# Autodesk Inventor assembly: #Spindexer
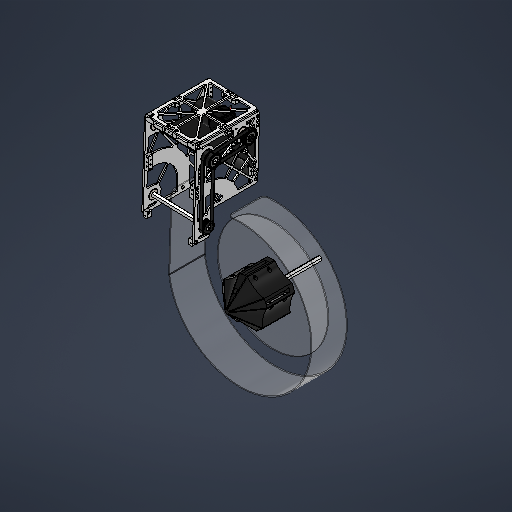
[picture p0: Inventor's stored thumbnail of the model, 512x512]
Saved by Autodesk Inventor 2026.1 (Build 301233020, 233B)
## iProperties
Created: 2026-02-05
Part Number: #Spindexer
Document SubType Name: Assembly
Designer: Owen L
Mass: 3778.08 g
Surface Area: 11708.6 cm^2
Volume: 3965.25 cm^3
Density: 0.952797 g/cm^3
Author: Owen L
## Documents named in this file (30)
- C:\Users\Owen\Documents\GitHub\2026-Robot-Mechanical\Spindexer\#Spindexer.iam
- C:\Users\Owen\Documents\GitHub\2026-Robot-Mechanical\Spindexer\3DPRINT,HUB.ipt
- C:\Users\Owen\Documents\GitHub\2026-Robot-Mechanical\Spindexer\3DPRINT,HUB,CONE.ipt
- C:\Users\Owen\Documents\GitHub\2026-Robot-Mechanical\Spindexer\PLATE,WALL.ipt
- C:\Users\Owen\Documents\GitHub\2026-Robot-Mechanical\Spindexer\PLATE,BOTTOM.ipt
- C:\Users\Owen\Documents\GitHub\2026-Robot-Mechanical\Spindexer\STOCK,HEX,SHAFT,HUB.ipt
- C:\Users\Owen\Documents\GitHub\2026-Robot-Mechanical\Spindexer\TEMP,BASE-SKETCH,TANGENT-OUT.ipt
- C:\Users\Owen\Documents\GitHub\2026-Robot-Mechanical\Spindexer\PLATE,KICKER,OUTSIDE.ipt
- C:\Users\Owen\Documents\GitHub\2026-Robot-Mechanical\Spindexer\3DPRINT,KICKER,RAMP.ipt
- C:\Users\Owen\Documents\GitHub\2026-Robot-Mechanical\Spindexer\PLATE,KICKER,INSIDE.ipt
- C:\Users\Owen\Documents\GitHub\2026-Robot-Mechanical\Spindexer\STOCK,HEX,SHAFT,KICKER,FRONT.ipt
- C:\Users\Owen\Documents\GitHub\2026-Robot-Mechanical\Spindexer\STOCK,HEX,SHAFT,KICKER,BACK.ipt
- C:\Users\Owen\Documents\GitHub\2026-Robot-Mechanical\#1_CAD Library\Power Transmission\Bearings\PURCHASED,HEX_BEARING.ipt
- C:\Users\Owen\Documents\GitHub\2026-Robot-Mechanical\#1_CAD Library\Power Transmission\VersaPlanetary\GEARBOX,VERSAPLANETARY,SINGLE-STAGE,HEX-SHAFT,0.5IN.ipt
- C:\Users\Owen\Documents\GitHub\2026-Robot-Mechanical\#1_CAD Library\Power Transmission\VersaPlanetary\ADAPTER,CIM-NEO,VERSAPLANETARY.ipt
- C:\Users\Owen\Documents\GitHub\2026-Robot-Mechanical\#1_CAD Library\Motors\MOTOR,REV,NEO,V1-1.ipt
- C:\Users\Owen\Documents\GitHub\2026-Robot-Mechanical\Spindexer\PLATE,NUT-BLOCK,3-LONG.ipt
- C:\Users\Owen\Documents\GitHub\2026-Robot-Mechanical\Spindexer\PLATE,NUT-BLOCK,2-LONG.ipt
- C:\Users\Owen\Documents\GitHub\2026-Robot-Mechanical\Spindexer\PLATE,NUT-BLOCK,1-LONG.ipt
- C:\Users\Owen\Documents\GitHub\2026-Robot-Mechanical\#1_CAD Library\Electronics\CONTROLS,SPARK_MAX.ipt
- C:\Users\Owen\Documents\GitHub\2026-Robot-Mechanical\Spindexer\3DPRINT,SPARK_MAX,MOUNT.ipt
- C:\Users\Owen\Documents\GitHub\2026-Robot-Mechanical\Spindexer\PLATE,KICKER,BACK.ipt
- C:\Users\Owen\Documents\GitHub\2026-Robot-Mechanical\Spindexer\PLATE,NUT-BLOCK,L-SHAPE.ipt
- C:\Users\Owen\Documents\GitHub\2026-Robot-Mechanical\Spindexer\3DPRINTED,PULLEY,21T,9mm.ipt
- C:\Users\Owen\Documents\GitHub\2026-Robot-Mechanical\#1_CAD Library\Power Transmission\Pulleys\PURCHASED,HTD5mm,24T,PULLEY.ipt
- C:\Users\Owen\Documents\GitHub\2026-Robot-Mechanical\Spindexer\STANDIN,BELT,70T,HTD5mm.ipt
- C:\Users\Owen\Documents\GitHub\2026-Robot-Mechanical\Spindexer\STANDIN,BELT,100T,HTD5mm.ipt
- C:\Users\Owen\Documents\GitHub\2026-Robot-Mechanical\#1_CAD Library\Building Materials\Fasteners\Bolts\PURCHASED,10-32x0.5in,BUTTONHEAD,BOLT.ipt
- C:\Users\Owen\Documents\GitHub\2026-Robot-Mechanical\#1_CAD Library\Building Materials\Fasteners\Nuts\PURCHASED,NYLOCK,10-32,NUT.ipt
- C:\Users\Owen\Documents\GitHub\2026-Robot-Mechanical\#1_CAD Library\Building Materials\Fasteners\Bolts\PURCHASED,10-32x0.625in,BUTTONHEAD,BOLT.ipt
## Components (90 placed, 29 different names)
1. 3DPRINT,HUB:1 — Mate:11, Mate:12, Mate:13, Mate:15, Mate:16, Mate:17, Flush:2, Mate:18, Mate:19, Mate:20
2. 3DPRINT,HUB,CONE:1 — Mate:11, Mate:12, Mate:13
3. PLATE,WALL:1 — Mate:32, Flush:7, Flush:8, Mate:42, Mate:43
4. PLATE,BOTTOM:1 — Mate:18, Mate:19, Mate:20, Mate:32, Flush:7
5. STOCK,HEX,SHAFT,HUB:1 — Mate:16, Mate:17, Flush:2
6. TEMP,BASE-SKETCH,TANGENT-OUT:1
7. PLATE,KICKER,OUTSIDE:1 — Mate:22, Mate:23, Mate:24, Mate:25, Flush:3, Flush:4, Flush:8, Insert:1, Insert:4, Mate:34, Mate:35, Mate:42, Insert:7, Insert:8, Insert:9, Insert:10, Insert:13, Insert:19, Insert:20, Flush:12, Mate:43, Insert:23, Insert:24, Insert:34, Insert:35, Insert:36, Insert:37, Insert:38, Insert:39, Insert:40, Insert:41, Insert:42, Insert:43, Insert:44, Insert:45, Insert:46, Insert:47, Insert:48, Insert:49, Insert:50, Insert:79, Insert:80, Insert:81, Insert:82
8. 3DPRINT,KICKER,RAMP:1 — Mate:22, Mate:23, Mate:24
9. PLATE,KICKER,INSIDE:1 — Mate:25, Flush:3, Flush:4, Insert:2, Insert:3, Mate:39, Mate:40, Mate:41, Insert:6, Insert:14, Insert:17, Insert:18, Insert:21, Insert:22, Insert:31, Insert:32, Insert:33, Mate:48, Mate:52, Insert:61, Insert:62, Insert:63, Insert:64, Insert:65, Insert:66, Insert:67, Insert:68, Insert:69, Insert:70, Insert:71, Insert:72, Insert:73, Insert:74, Insert:75, Insert:76, Insert:77, Insert:78
10. STOCK,HEX,SHAFT,KICKER,FRONT:1 — Mate:34, Mate:45, Flush:15
11. STOCK,HEX,SHAFT,KICKER,BACK:1 — Mate:35, Mate:46, Mate:47, Flush:14
12. PURCHASED,HEX_BEARING:1 — Insert:1, Flush:15
13. PURCHASED,HEX_BEARING:2 — Insert:2, Mate:50
14. PURCHASED,HEX_BEARING:3 — Insert:3, Mate:49
15. PURCHASED,HEX_BEARING:4 — Insert:4, Flush:14
16. GEARBOX,VERSAPLANETARY,SINGLE-STAGE,HEX-SHAFT,0.5IN:1 — Mate:36, Mate:37, Mate:38, Mate:39, Mate:40, Mate:41, Mate:53
17. ADAPTER,CIM-NEO,VERSAPLANETARY:1 — Mate:36, Mate:37, Mate:38, Insert:5
18. MOTOR,REV,NEO,V1-1:1 — Insert:5
19. PLATE,NUT-BLOCK,3-LONG:1 — Insert:6
20. PLATE,NUT-BLOCK,3-LONG:2 — Insert:9, Insert:10
21. PLATE,NUT-BLOCK,3-LONG:3 — Insert:7, Insert:8
22. PLATE,NUT-BLOCK,1-LONG:1 — Insert:13, Flush:11, Flush:12
23. PLATE,NUT-BLOCK,1-LONG:2 — Insert:14, Flush:11
24. PLATE,NUT-BLOCK,3-LONG:4 — Insert:17, Insert:18
25. PLATE,NUT-BLOCK,3-LONG:5 — Insert:19, Insert:20
26. CONTROLS,SPARK_MAX:1
27. 3DPRINT,SPARK_MAX,MOUNT:1
28. PLATE,KICKER,BACK:1 — Mate:44, Insert:25, Insert:26, Insert:27, Insert:28, Insert:29, Insert:30, Insert:51, Insert:52, Insert:53, Insert:54, Insert:55, Insert:56, Insert:57, Insert:58, Insert:59, Insert:60
29. PLATE,NUT-BLOCK,2-LONG:2 — Insert:21, Insert:22, Mate:44, Insert:26
30. PLATE,NUT-BLOCK,2-LONG:3 — Insert:23, Insert:24, Insert:25
31. PLATE,NUT-BLOCK,3-LONG:6 — Insert:27, Insert:28
32. PLATE,NUT-BLOCK,3-LONG:7 — Insert:29, Insert:30
33. PLATE,NUT-BLOCK,3-LONG:8 — Insert:31, Insert:32
34. PLATE,NUT-BLOCK,L-SHAPE:1 — Insert:33
35. PLATE,NUT-BLOCK,L-SHAPE:2 — Insert:34
36. 3DPRINTED,PULLEY,21T,9mm:1 — Mate:46, Mate:49, Mate:51, Mate:55, Mate:58
37. 3DPRINTED,PULLEY,21T,9mm:2 — Mate:45, Mate:50, Mate:54
38. PURCHASED,HEX_BEARING:5 — Mate:52, Mate:53
39. PURCHASED,HTD5mm,24T,PULLEY:1 — Mate:47, Mate:51, Flush:13, Mate:57
40. PURCHASED,HTD5mm,24T,PULLEY:2 — Mate:48, Flush:13, Mate:56
41. STANDIN,BELT,70T,HTD5mm:1 — Mate:56, Mate:57
42. STANDIN,BELT,100T,HTD5mm:1 — Mate:54, Mate:55, Mate:58
43. PURCHASED,10-32x0.5in,BUTTONHEAD,BOLT:1 — Insert:48
44. PURCHASED,NYLOCK,10-32,NUT:1 — Insert:81
45. PURCHASED,10-32x0.625in,BUTTONHEAD,BOLT:1 — Insert:35
46. PURCHASED,10-32x0.625in,BUTTONHEAD,BOLT:2 — Insert:36
47. PURCHASED,10-32x0.625in,BUTTONHEAD,BOLT:3 — Insert:37
48. PURCHASED,10-32x0.625in,BUTTONHEAD,BOLT:4 — Insert:38
49. PURCHASED,10-32x0.625in,BUTTONHEAD,BOLT:5 — Insert:39
50. PURCHASED,10-32x0.625in,BUTTONHEAD,BOLT:6 — Insert:40
51. PURCHASED,10-32x0.625in,BUTTONHEAD,BOLT:7 — Insert:41
52. PURCHASED,10-32x0.625in,BUTTONHEAD,BOLT:8 — Insert:42
53. PURCHASED,10-32x0.625in,BUTTONHEAD,BOLT:9 — Insert:43
54. PURCHASED,10-32x0.625in,BUTTONHEAD,BOLT:10 — Insert:44
55. PURCHASED,10-32x0.625in,BUTTONHEAD,BOLT:11 — Insert:45
56. PURCHASED,10-32x0.625in,BUTTONHEAD,BOLT:12 — Insert:46
57. PURCHASED,10-32x0.625in,BUTTONHEAD,BOLT:13 — Insert:47
58. PURCHASED,10-32x0.625in,BUTTONHEAD,BOLT:14 — Insert:51
59. PURCHASED,10-32x0.625in,BUTTONHEAD,BOLT:15 — Insert:52
60. PURCHASED,10-32x0.625in,BUTTONHEAD,BOLT:16 — Insert:53
61. PURCHASED,10-32x0.625in,BUTTONHEAD,BOLT:17 — Insert:54
62. PURCHASED,10-32x0.625in,BUTTONHEAD,BOLT:18 — Insert:55
63. PURCHASED,10-32x0.5in,BUTTONHEAD,BOLT:2 — Insert:49
64. PURCHASED,10-32x0.5in,BUTTONHEAD,BOLT:3 — Insert:50
65. PURCHASED,10-32x0.625in,BUTTONHEAD,BOLT:19 — Insert:59
66. PURCHASED,10-32x0.625in,BUTTONHEAD,BOLT:20 — Insert:58
67. PURCHASED,10-32x0.625in,BUTTONHEAD,BOLT:21 — Insert:56
68. PURCHASED,10-32x0.625in,BUTTONHEAD,BOLT:22 — Insert:60
69. PURCHASED,10-32x0.625in,BUTTONHEAD,BOLT:23 — Insert:57
70. PURCHASED,10-32x0.625in,BUTTONHEAD,BOLT:24 — Insert:61
71. PURCHASED,10-32x0.625in,BUTTONHEAD,BOLT:25 — Insert:62
72. PURCHASED,10-32x0.625in,BUTTONHEAD,BOLT:26 — Insert:63
73. PURCHASED,10-32x0.625in,BUTTONHEAD,BOLT:27 — Insert:64
74. PURCHASED,10-32x0.625in,BUTTONHEAD,BOLT:28 — Insert:65
75. PURCHASED,10-32x0.625in,BUTTONHEAD,BOLT:29 — Insert:66
76. PURCHASED,10-32x0.625in,BUTTONHEAD,BOLT:30 — Insert:67
77. PURCHASED,10-32x0.625in,BUTTONHEAD,BOLT:31 — Insert:68
78. PURCHASED,10-32x0.625in,BUTTONHEAD,BOLT:32 — Insert:69
79. PURCHASED,10-32x0.625in,BUTTONHEAD,BOLT:33 — Insert:70
80. PURCHASED,10-32x0.625in,BUTTONHEAD,BOLT:34 — Insert:73
81. PURCHASED,10-32x0.625in,BUTTONHEAD,BOLT:35 — Insert:72
82. PURCHASED,10-32x0.625in,BUTTONHEAD,BOLT:36 — Insert:71
83. PURCHASED,10-32x0.5in,BUTTONHEAD,BOLT:4 — Insert:74
84. PURCHASED,10-32x0.5in,BUTTONHEAD,BOLT:5 — Insert:76
85. PURCHASED,10-32x0.5in,BUTTONHEAD,BOLT:6 — Insert:75
86. PURCHASED,10-32x0.5in,BUTTONHEAD,BOLT:7 — Insert:77
87. PURCHASED,10-32x0.5in,BUTTONHEAD,BOLT:8 — Insert:78
88. PURCHASED,10-32x0.5in,BUTTONHEAD,BOLT:9 — Insert:79
89. PURCHASED,10-32x0.5in,BUTTONHEAD,BOLT:10 — Insert:80
90. PURCHASED,NYLOCK,10-32,NUT:2 — Insert:82
## Relationships (127: Insert 78, Mate 39, Flush 10)
- Mate:11: 3DPRINT,HUB:1 ↔ 3DPRINT,HUB,CONE:1
- Mate:12: 3DPRINT,HUB:1 ↔ 3DPRINT,HUB,CONE:1
- Mate:13: 3DPRINT,HUB:1 ↔ 3DPRINT,HUB,CONE:1
- Mate:15: 3DPRINT,HUB:1
- Mate:16: 3DPRINT,HUB:1 ↔ STOCK,HEX,SHAFT,HUB:1
- Mate:17: 3DPRINT,HUB:1 ↔ STOCK,HEX,SHAFT,HUB:1
- Flush:2 (-12.7 mm): 3DPRINT,HUB:1 ↔ STOCK,HEX,SHAFT,HUB:1
- Mate:18: 3DPRINT,HUB:1 ↔ PLATE,BOTTOM:1
- Mate:19: 3DPRINT,HUB:1 ↔ PLATE,BOTTOM:1
- Mate:20: 3DPRINT,HUB:1 ↔ PLATE,BOTTOM:1
- Mate:22: PLATE,KICKER,OUTSIDE:1 ↔ 3DPRINT,KICKER,RAMP:1
- Mate:23: PLATE,KICKER,OUTSIDE:1 ↔ 3DPRINT,KICKER,RAMP:1
- Mate:24: PLATE,KICKER,OUTSIDE:1 ↔ 3DPRINT,KICKER,RAMP:1
- Mate:25 (158.75 mm): PLATE,KICKER,OUTSIDE:1 ↔ PLATE,KICKER,INSIDE:1
- Flush:3: PLATE,KICKER,OUTSIDE:1 ↔ PLATE,KICKER,INSIDE:1
- Flush:4: PLATE,KICKER,OUTSIDE:1 ↔ PLATE,KICKER,INSIDE:1
- Mate:32: PLATE,WALL:1 ↔ PLATE,BOTTOM:1
- Flush:7 (-6.35 mm): PLATE,WALL:1 ↔ PLATE,BOTTOM:1
- Flush:8: PLATE,WALL:1 ↔ PLATE,KICKER,OUTSIDE:1
- Insert:1: PLATE,KICKER,OUTSIDE:1 ↔ PURCHASED,HEX_BEARING:1
- Insert:2: PLATE,KICKER,INSIDE:1 ↔ PURCHASED,HEX_BEARING:2
- Insert:3: PLATE,KICKER,INSIDE:1 ↔ PURCHASED,HEX_BEARING:3
- Insert:4: PLATE,KICKER,OUTSIDE:1 ↔ PURCHASED,HEX_BEARING:4
- Mate:34: PLATE,KICKER,OUTSIDE:1 ↔ STOCK,HEX,SHAFT,KICKER,FRONT:1
- Mate:35: PLATE,KICKER,OUTSIDE:1 ↔ STOCK,HEX,SHAFT,KICKER,BACK:1
- Mate:36: GEARBOX,VERSAPLANETARY,SINGLE-STAGE,HEX-SHAFT,0.5IN:1 ↔ ADAPTER,CIM-NEO,VERSAPLANETARY:1
- Mate:37: GEARBOX,VERSAPLANETARY,SINGLE-STAGE,HEX-SHAFT,0.5IN:1 ↔ ADAPTER,CIM-NEO,VERSAPLANETARY:1
- Mate:38: GEARBOX,VERSAPLANETARY,SINGLE-STAGE,HEX-SHAFT,0.5IN:1 ↔ ADAPTER,CIM-NEO,VERSAPLANETARY:1
- Insert:5: ADAPTER,CIM-NEO,VERSAPLANETARY:1 ↔ MOTOR,REV,NEO,V1-1:1
- Mate:39: PLATE,KICKER,INSIDE:1 ↔ GEARBOX,VERSAPLANETARY,SINGLE-STAGE,HEX-SHAFT,0.5IN:1
- Mate:40: PLATE,KICKER,INSIDE:1 ↔ GEARBOX,VERSAPLANETARY,SINGLE-STAGE,HEX-SHAFT,0.5IN:1
- Mate:41: PLATE,KICKER,INSIDE:1 ↔ GEARBOX,VERSAPLANETARY,SINGLE-STAGE,HEX-SHAFT,0.5IN:1
- Mate:42: PLATE,WALL:1 ↔ PLATE,KICKER,OUTSIDE:1
- Insert:6: PLATE,KICKER,INSIDE:1 ↔ PLATE,NUT-BLOCK,3-LONG:1
- Insert:7: PLATE,KICKER,OUTSIDE:1 ↔ PLATE,NUT-BLOCK,3-LONG:3
- Insert:8: PLATE,KICKER,OUTSIDE:1 ↔ PLATE,NUT-BLOCK,3-LONG:3
- Insert:9: PLATE,KICKER,OUTSIDE:1 ↔ PLATE,NUT-BLOCK,3-LONG:2
- Insert:10: PLATE,KICKER,OUTSIDE:1 ↔ PLATE,NUT-BLOCK,3-LONG:2
- Insert:13: PLATE,KICKER,OUTSIDE:1 ↔ PLATE,NUT-BLOCK,1-LONG:1
- Insert:14: PLATE,KICKER,INSIDE:1 ↔ PLATE,NUT-BLOCK,1-LONG:2
- Insert:17: PLATE,KICKER,INSIDE:1 ↔ PLATE,NUT-BLOCK,3-LONG:4
- Insert:18: PLATE,KICKER,INSIDE:1 ↔ PLATE,NUT-BLOCK,3-LONG:4
- Insert:19: PLATE,KICKER,OUTSIDE:1 ↔ PLATE,NUT-BLOCK,3-LONG:5
- Insert:20: PLATE,KICKER,OUTSIDE:1 ↔ PLATE,NUT-BLOCK,3-LONG:5
- Flush:11: PLATE,NUT-BLOCK,1-LONG:1 ↔ PLATE,NUT-BLOCK,1-LONG:2
- Flush:12: PLATE,KICKER,OUTSIDE:1 ↔ PLATE,NUT-BLOCK,1-LONG:1
- Mate:43 (-25.4 mm): PLATE,WALL:1 ↔ PLATE,KICKER,OUTSIDE:1
- Insert:21: PLATE,KICKER,INSIDE:1 ↔ PLATE,NUT-BLOCK,2-LONG:2
- Insert:22: PLATE,KICKER,INSIDE:1 ↔ PLATE,NUT-BLOCK,2-LONG:2
- Insert:23: PLATE,KICKER,OUTSIDE:1 ↔ PLATE,NUT-BLOCK,2-LONG:3
- Insert:24: PLATE,KICKER,OUTSIDE:1 ↔ PLATE,NUT-BLOCK,2-LONG:3
- Mate:44: PLATE,KICKER,BACK:1 ↔ PLATE,NUT-BLOCK,2-LONG:2
- Insert:25: PLATE,KICKER,BACK:1 ↔ PLATE,NUT-BLOCK,2-LONG:3
- Insert:26: PLATE,KICKER,BACK:1 ↔ PLATE,NUT-BLOCK,2-LONG:2
- Insert:27: PLATE,KICKER,BACK:1 ↔ PLATE,NUT-BLOCK,3-LONG:6
- Insert:28: PLATE,KICKER,BACK:1 ↔ PLATE,NUT-BLOCK,3-LONG:6
- Insert:29: PLATE,KICKER,BACK:1 ↔ PLATE,NUT-BLOCK,3-LONG:7
- Insert:30: PLATE,KICKER,BACK:1 ↔ PLATE,NUT-BLOCK,3-LONG:7
- Insert:31: PLATE,KICKER,INSIDE:1 ↔ PLATE,NUT-BLOCK,3-LONG:8
- Insert:32: PLATE,KICKER,INSIDE:1 ↔ PLATE,NUT-BLOCK,3-LONG:8
- Insert:33: PLATE,KICKER,INSIDE:1 ↔ PLATE,NUT-BLOCK,L-SHAPE:1
- Insert:34: PLATE,KICKER,OUTSIDE:1 ↔ PLATE,NUT-BLOCK,L-SHAPE:2
- Mate:45: STOCK,HEX,SHAFT,KICKER,FRONT:1 ↔ 3DPRINTED,PULLEY,21T,9mm:2
- Mate:46: STOCK,HEX,SHAFT,KICKER,BACK:1 ↔ 3DPRINTED,PULLEY,21T,9mm:1
- Mate:47: STOCK,HEX,SHAFT,KICKER,BACK:1 ↔ PURCHASED,HTD5mm,24T,PULLEY:1
- Mate:48: PLATE,KICKER,INSIDE:1 ↔ PURCHASED,HTD5mm,24T,PULLEY:2
- Mate:49: PURCHASED,HEX_BEARING:3 ↔ 3DPRINTED,PULLEY,21T,9mm:1
- Mate:50: PURCHASED,HEX_BEARING:2 ↔ 3DPRINTED,PULLEY,21T,9mm:2
- Mate:51: 3DPRINTED,PULLEY,21T,9mm:1 ↔ PURCHASED,HTD5mm,24T,PULLEY:1
- Flush:13: PURCHASED,HTD5mm,24T,PULLEY:1 ↔ PURCHASED,HTD5mm,24T,PULLEY:2
- Flush:14: STOCK,HEX,SHAFT,KICKER,BACK:1 ↔ PURCHASED,HEX_BEARING:4
- Flush:15: STOCK,HEX,SHAFT,KICKER,FRONT:1 ↔ PURCHASED,HEX_BEARING:1
- Mate:52: PLATE,KICKER,INSIDE:1 ↔ PURCHASED,HEX_BEARING:5
- Mate:53: GEARBOX,VERSAPLANETARY,SINGLE-STAGE,HEX-SHAFT,0.5IN:1 ↔ PURCHASED,HEX_BEARING:5
- Mate:54: 3DPRINTED,PULLEY,21T,9mm:2 ↔ STANDIN,BELT,100T,HTD5mm:1
- Mate:55: 3DPRINTED,PULLEY,21T,9mm:1 ↔ STANDIN,BELT,100T,HTD5mm:1
- Mate:56: PURCHASED,HTD5mm,24T,PULLEY:2 ↔ STANDIN,BELT,70T,HTD5mm:1
- Mate:57: PURCHASED,HTD5mm,24T,PULLEY:1 ↔ STANDIN,BELT,70T,HTD5mm:1
- Mate:58: 3DPRINTED,PULLEY,21T,9mm:1 ↔ STANDIN,BELT,100T,HTD5mm:1
- Insert:35: PLATE,KICKER,OUTSIDE:1 ↔ PURCHASED,10-32x0.625in,BUTTONHEAD,BOLT:1
- Insert:36: PLATE,KICKER,OUTSIDE:1 ↔ PURCHASED,10-32x0.625in,BUTTONHEAD,BOLT:2
- Insert:37: PLATE,KICKER,OUTSIDE:1 ↔ PURCHASED,10-32x0.625in,BUTTONHEAD,BOLT:3
- Insert:38: PLATE,KICKER,OUTSIDE:1 ↔ PURCHASED,10-32x0.625in,BUTTONHEAD,BOLT:4
- Insert:39: PLATE,KICKER,OUTSIDE:1 ↔ PURCHASED,10-32x0.625in,BUTTONHEAD,BOLT:5
- Insert:40: PLATE,KICKER,OUTSIDE:1 ↔ PURCHASED,10-32x0.625in,BUTTONHEAD,BOLT:6
- Insert:41: PLATE,KICKER,OUTSIDE:1 ↔ PURCHASED,10-32x0.625in,BUTTONHEAD,BOLT:7
- Insert:42: PLATE,KICKER,OUTSIDE:1 ↔ PURCHASED,10-32x0.625in,BUTTONHEAD,BOLT:8
- Insert:43: PLATE,KICKER,OUTSIDE:1 ↔ PURCHASED,10-32x0.625in,BUTTONHEAD,BOLT:9
- Insert:44: PLATE,KICKER,OUTSIDE:1 ↔ PURCHASED,10-32x0.625in,BUTTONHEAD,BOLT:10
- Insert:45: PLATE,KICKER,OUTSIDE:1 ↔ PURCHASED,10-32x0.625in,BUTTONHEAD,BOLT:11
- Insert:46: PLATE,KICKER,OUTSIDE:1 ↔ PURCHASED,10-32x0.625in,BUTTONHEAD,BOLT:12
- Insert:47: PLATE,KICKER,OUTSIDE:1 ↔ PURCHASED,10-32x0.625in,BUTTONHEAD,BOLT:13
- Insert:48: PLATE,KICKER,OUTSIDE:1 ↔ PURCHASED,10-32x0.5in,BUTTONHEAD,BOLT:1
- Insert:49: PLATE,KICKER,OUTSIDE:1 ↔ PURCHASED,10-32x0.5in,BUTTONHEAD,BOLT:2
- Insert:50: PLATE,KICKER,OUTSIDE:1 ↔ PURCHASED,10-32x0.5in,BUTTONHEAD,BOLT:3
- Insert:51: PLATE,KICKER,BACK:1 ↔ PURCHASED,10-32x0.625in,BUTTONHEAD,BOLT:14
- Insert:52: PLATE,KICKER,BACK:1 ↔ PURCHASED,10-32x0.625in,BUTTONHEAD,BOLT:15
- Insert:53: PLATE,KICKER,BACK:1 ↔ PURCHASED,10-32x0.625in,BUTTONHEAD,BOLT:16
- Insert:54: PLATE,KICKER,BACK:1 ↔ PURCHASED,10-32x0.625in,BUTTONHEAD,BOLT:17
- Insert:55: PLATE,KICKER,BACK:1 ↔ PURCHASED,10-32x0.625in,BUTTONHEAD,BOLT:18
- Insert:56: PLATE,KICKER,BACK:1 ↔ PURCHASED,10-32x0.625in,BUTTONHEAD,BOLT:21
- Insert:57: PLATE,KICKER,BACK:1 ↔ PURCHASED,10-32x0.625in,BUTTONHEAD,BOLT:23
- Insert:58: PLATE,KICKER,BACK:1 ↔ PURCHASED,10-32x0.625in,BUTTONHEAD,BOLT:20
- Insert:59: PLATE,KICKER,BACK:1 ↔ PURCHASED,10-32x0.625in,BUTTONHEAD,BOLT:19
- Insert:60: PLATE,KICKER,BACK:1 ↔ PURCHASED,10-32x0.625in,BUTTONHEAD,BOLT:22
- Insert:61: PLATE,KICKER,INSIDE:1 ↔ PURCHASED,10-32x0.625in,BUTTONHEAD,BOLT:24
- Insert:62: PLATE,KICKER,INSIDE:1 ↔ PURCHASED,10-32x0.625in,BUTTONHEAD,BOLT:25
- Insert:63: PLATE,KICKER,INSIDE:1 ↔ PURCHASED,10-32x0.625in,BUTTONHEAD,BOLT:26
- Insert:64: PLATE,KICKER,INSIDE:1 ↔ PURCHASED,10-32x0.625in,BUTTONHEAD,BOLT:27
- Insert:65: PLATE,KICKER,INSIDE:1 ↔ PURCHASED,10-32x0.625in,BUTTONHEAD,BOLT:28
- Insert:66: PLATE,KICKER,INSIDE:1 ↔ PURCHASED,10-32x0.625in,BUTTONHEAD,BOLT:29
- Insert:67: PLATE,KICKER,INSIDE:1 ↔ PURCHASED,10-32x0.625in,BUTTONHEAD,BOLT:30
- Insert:68: PLATE,KICKER,INSIDE:1 ↔ PURCHASED,10-32x0.625in,BUTTONHEAD,BOLT:31
- Insert:69: PLATE,KICKER,INSIDE:1 ↔ PURCHASED,10-32x0.625in,BUTTONHEAD,BOLT:32
- Insert:70: PLATE,KICKER,INSIDE:1 ↔ PURCHASED,10-32x0.625in,BUTTONHEAD,BOLT:33
- Insert:71: PLATE,KICKER,INSIDE:1 ↔ PURCHASED,10-32x0.625in,BUTTONHEAD,BOLT:36
- Insert:72: PLATE,KICKER,INSIDE:1 ↔ PURCHASED,10-32x0.625in,BUTTONHEAD,BOLT:35
- Insert:73: PLATE,KICKER,INSIDE:1 ↔ PURCHASED,10-32x0.625in,BUTTONHEAD,BOLT:34
- Insert:74: PLATE,KICKER,INSIDE:1 ↔ PURCHASED,10-32x0.5in,BUTTONHEAD,BOLT:4
- Insert:75: PLATE,KICKER,INSIDE:1 ↔ PURCHASED,10-32x0.5in,BUTTONHEAD,BOLT:6
- Insert:76: PLATE,KICKER,INSIDE:1 ↔ PURCHASED,10-32x0.5in,BUTTONHEAD,BOLT:5
- Insert:77: PLATE,KICKER,INSIDE:1 ↔ PURCHASED,10-32x0.5in,BUTTONHEAD,BOLT:7
- Insert:78: PLATE,KICKER,INSIDE:1 ↔ PURCHASED,10-32x0.5in,BUTTONHEAD,BOLT:8
- Insert:79: PLATE,KICKER,OUTSIDE:1 ↔ PURCHASED,10-32x0.5in,BUTTONHEAD,BOLT:9
- Insert:80: PLATE,KICKER,OUTSIDE:1 ↔ PURCHASED,10-32x0.5in,BUTTONHEAD,BOLT:10
- Insert:81: PLATE,KICKER,OUTSIDE:1 ↔ PURCHASED,NYLOCK,10-32,NUT:1
- Insert:82: PLATE,KICKER,OUTSIDE:1 ↔ PURCHASED,NYLOCK,10-32,NUT:2
